# Autodesk Inventor assembly: LiDAR
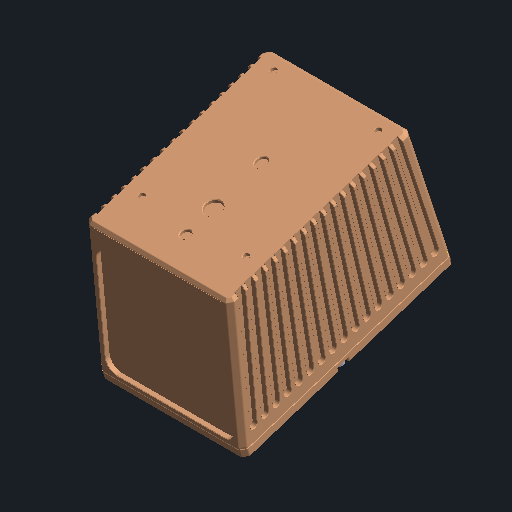
[picture p0: Inventor's stored thumbnail of the model, 512x512]
Saved by Autodesk Inventor 2022 (Build 260153000, 153)
## iProperties
Part Number: LiDAR
Document SubType Name: Ensamblaje
Designer: seb_0
Author: seb_0
## Documents named in this file (3)
- D:\Documentos\15.PUCP_2021-2\[PDM] Proyecto de Diseño Mecatrónico\ProyectoGIT\ProyectoRobotPallet\LiDAR\LiDAR.iam
- D:\Documentos\15.PUCP_2021-2\[PDM] Proyecto de Diseño Mecatrónico\ProyectoGIT\ProyectoRobotPallet\LiDAR\Soporte_LíDAR.ipt
- D:\Documentos\15.PUCP_2021-2\[PDM] Proyecto de Diseño Mecatrónico\ProyectoGIT\ProyectoRobotPallet\LiDAR\Livox Mid-70.ipt
## Components (2 placed, 2 different names)
1. Soporte_LíDAR:1 — Coincidencia:1, Coincidencia:2, Coincidencia:3, Coincidencia:4, Coincidencia:5
2. Livox Mid-70:1 — Coincidencia:3, Coincidencia:4, Coincidencia:5
## Relationships (5: Mate 5)
- Coincidencia:1 [Mate]: Soporte_LíDAR:1
- Coincidencia:2 [Mate]: Soporte_LíDAR:1
- Coincidencia:3 [Mate]: Soporte_LíDAR:1 ↔ Livox Mid-70:1
- Coincidencia:4 [Mate]: Soporte_LíDAR:1 ↔ Livox Mid-70:1
- Coincidencia:5 [Mate]: Soporte_LíDAR:1 ↔ Livox Mid-70:1
